# Autodesk Inventor assembly: WR-LEN-AS
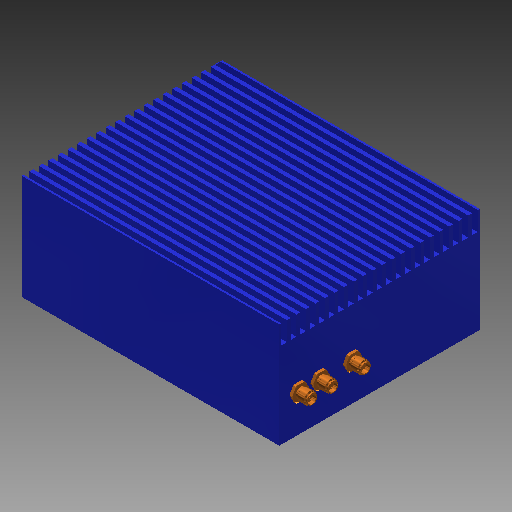
[picture p0: Inventor's stored thumbnail of the model, 512x512]
Saved by Autodesk Inventor 2018 (Build 220112000, 112)
## iProperties
Created: 2022-04-20
Part Number: WR-LEN-AS
Document SubType Name: Assembly
Designer: pollak
Author: pollak
## Documents named in this file (4)
- C:\Users\pollak\ownCloud\Inventor\ATA_2019\NRDZ-Sensor_2022\WR-LEN-AS.iam
- C:\Users\pollak\ownCloud\Inventor\ATA_2019\NRDZ-Sensor_2022\WR-LEN-base.ipt
- C:\Users\pollak\ownCloud\Inventor\ATA_2019\Shared_Parts\RJ45-connector\xb5prj45.iam
- C:\Users\pollak\ownCloud\Inventor\ATA_2019\Shared_Parts\r125720001.ipt
## Components (5 placed, 3 different names)
1. WR-LEN-base:1 — Mate:1, Flush:1, Flush:2, Mate:2, Mate:3, Mate:4, Flush:3, Flush:4, Flush:5, Tangent:1, Tangent:2, Tangent:3
2. xb5prj45:1 [sub-assembly] — Mate:1, Flush:1, Flush:2
3. r125720001:1 — Mate:2, Flush:3, Tangent:1
4. r125720001:2 — Mate:3, Flush:5, Tangent:2
5. r125720001:3 — Mate:4, Flush:4, Tangent:3
## Relationships (12: Flush 5, Mate 4, Tangent 3)
- Mate:1: WR-LEN-base:1 ↔ xb5prj45:1
- Flush:1 (40 mm): WR-LEN-base:1 ↔ xb5prj45:1
- Flush:2 (59 mm): WR-LEN-base:1 ↔ xb5prj45:1
- Mate:2: WR-LEN-base:1 ↔ r125720001:1
- Mate:3: WR-LEN-base:1 ↔ r125720001:2
- Mate:4: WR-LEN-base:1 ↔ r125720001:3
- Flush:3 (16 mm): WR-LEN-base:1 ↔ r125720001:1
- Flush:4 (16 mm): WR-LEN-base:1 ↔ r125720001:3
- Flush:5 (16 mm): WR-LEN-base:1 ↔ r125720001:2
- Tangent:1 (5 mm): WR-LEN-base:1 ↔ r125720001:1
- Tangent:2 (16 mm): WR-LEN-base:1 ↔ r125720001:2
- Tangent:3 (33 mm): WR-LEN-base:1 ↔ r125720001:3
